# Autodesk Inventor assembly: Montagem1
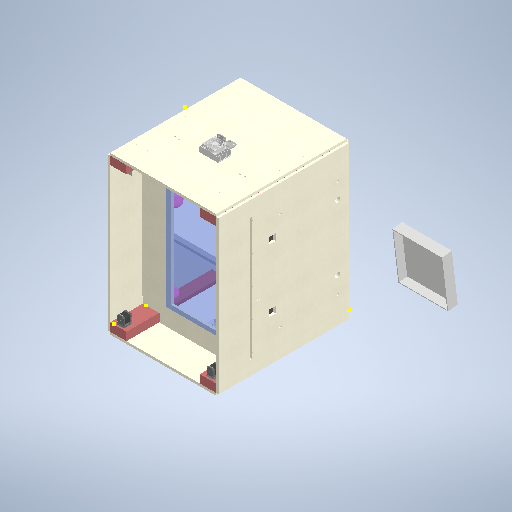
[picture p0: Inventor's stored thumbnail of the model, 512x512]
Saved by Autodesk Inventor 2025.1 (Build 291241000, 241)
## iProperties
Created: 2024-11-05
Part Number: Montagem1
Document SubType Name: Assembly
Designer: pedro
Author: pedro
## Documents named in this file (10)
- C:\Users\pedro\Documents\1-CoisasSerias\UTFPR\2024-2\Oficina\Estrutura\Montagem1 - Copia.iam
- C:\Users\pedro\Documents\1-CoisasSerias\UTFPR\2024-2\Oficina\Estrutura\estrutura2.ipt
- C:\Users\pedro\Documents\1-CoisasSerias\UTFPR\2024-2\Oficina\Estrutura\Pecas Prontas\Fan\Generic 7015 axial fan simplified\Generic 7015 axial fan simplified\cooler 40x40.ipt
- C:\Users\pedro\Documents\1-CoisasSerias\UTFPR\2024-2\Oficina\Estrutura\Pecas Prontas\Let light\Soquete\Soquete para lâmpada E27 MT-2302 - DECORLUX\Soquete para lâmpada E27 MT-2302 - DECORLUX\Soquete para lâmpad.iam
- C:\Users\pedro\Documents\1-CoisasSerias\UTFPR\2024-2\Oficina\Estrutura\step mother.iam
- C:\Users\pedro\Documents\1-CoisasSerias\UTFPR\2024-2\Oficina\Estrutura\Pecas Prontas\peltier\75W Peltier Air Cooler Kit 12V (TEC1-12706) - WiMas\75W Peltier Air Cooler Kit 12V (TEC1-12706) - WiMas\75W Peltier A.iam
- C:\Users\pedro\Documents\1-CoisasSerias\UTFPR\2024-2\Oficina\Estrutura\Pecas Prontas\peltier\step\L Bracket\L Bracket\L Bracket.ipt
- C:\Users\pedro\Documents\1-CoisasSerias\UTFPR\2024-2\Oficina\Estrutura\Pecas Prontas\reservatorio.ipt
- C:\Users\pedro\Documents\1-CoisasSerias\UTFPR\2024-2\Oficina\Estrutura\Pecas Prontas\vaso.ipt
- C:\Users\pedro\Documents\1-CoisasSerias\UTFPR\2024-2\Oficina\Estrutura\Pecas Prontas\temp\nema17-mounting-l-bracket-1.snapshot.2\NEMA17MountingLBracket.ipt
## Components (27 placed, 9 different names)
1. estrutura2:1 — Alinhado:1, Ângulo:1, Alinhado:2, Alinhado:3, Coincidente:1, Ângulo:2, Coincidente:2, Ângulo:3, Coincidente:12, Coincidente:13, Coincidente:14, Coincidente:15, Coincidente:18, Coincidente:19, Coincidente:20, Coincidente:21, Coincidente:22, Coincidente:26, Coincidente:27, Coincidente:28, Coincidente:29, Coincidente:31, Coincidente:32, Coincidente:33, Coincidente:34, Coincidente:35, Coincidente:36, Coincidente:37, Coincidente:38, Coincidente:39, Coincidente:40, Coincidente:41, Coincidente:42, Coincidente:43, Coincidente:44, Coincidente:45, Coincidente:46, Coincidente:47, Coincidente:48, Coincidente:49, Coincidente:50, Coincidente:51, Coincidente:52, Coincidente:53, Coincidente:54, Coincidente:55, Coincidente:56, Coincidente:57, Coincidente:58, Coincidente:59
2. cooler 40x40:1 — Alinhado:1, Ângulo:1, Alinhado:2, Alinhado:3
3. cooler 40x40:2
4. cooler 40x40:3
5. cooler 40x40:4
6. Soquete para lâmpad:2 [sub-assembly] — Coincidente:38, Coincidente:39
7. Soquete para lâmpad:3 [sub-assembly] — Coincidente:40, Coincidente:41
8. Soquete para lâmpad:4 [sub-assembly] — Coincidente:36, Coincidente:37
9. Soquete para lâmpad:8 [sub-assembly] — Coincidente:12, Coincidente:13, Coincidente:45
10. Soquete para lâmpad:9 [sub-assembly] — Coincidente:14, Coincidente:15, Coincidente:44
11. Soquete para lâmpad:10 [sub-assembly] — Coincidente:42, Coincidente:43
12. step mother:1 [sub-assembly] — Coincidente:18, Coincidente:19, Coincidente:20, Coincidente:21, Coincidente:22
13. step mother:3 [sub-assembly] — Coincidente:52
14. 75W Peltier A:1 [sub-assembly] — Coincidente:26, Coincidente:27
15. 75W Peltier A:2 [sub-assembly] — Coincidente:28, Coincidente:29, Coincidente:30
16. L Bracket:1 — Coincidente:30, Coincidente:31
17. L Bracket:2 — Coincidente:32
18. reservatorio:1
19. vaso:1 — Coincidente:33, Coincidente:34, Coincidente:35
20. vaso:2
21. L Bracket:3 — Coincidente:46
22. L Bracket:4 — Coincidente:47, Coincidente:48, Coincidente:49
23. L Bracket:5 — Coincidente:50
24. L Bracket:6 — Coincidente:51
25. step mother:4 [sub-assembly] — Coincidente:53
26. NEMA17MountingLBracket:1 — Coincidente:54, Coincidente:55, Coincidente:56
27. NEMA17MountingLBracket:2 — Coincidente:57, Coincidente:58, Coincidente:59
## Relationships (51: Mate 45, Flush 3, Angle 3)
- Alinhado:1 [Flush] (15 mm): estrutura2:1 ↔ cooler 40x40:1
- Ângulo:1 [Angle] (0 deg): estrutura2:1 ↔ cooler 40x40:1
- Alinhado:2 [Flush] (270 mm): estrutura2:1 ↔ cooler 40x40:1
- Alinhado:3 [Flush] (310 mm): estrutura2:1 ↔ cooler 40x40:1
- Coincidente:1 [Mate]: estrutura2:1
- Ângulo:2 [Angle] (0 deg): estrutura2:1
- Coincidente:2 [Mate]: estrutura2:1
- Ângulo:3 [Angle] (0 deg): estrutura2:1
- Coincidente:12 [Mate]: estrutura2:1 ↔ Soquete para lâmpad:8
- Coincidente:13 [Mate]: estrutura2:1 ↔ Soquete para lâmpad:8
- Coincidente:14 [Mate]: estrutura2:1 ↔ Soquete para lâmpad:9
- Coincidente:15 [Mate]: estrutura2:1 ↔ Soquete para lâmpad:9
- Coincidente:18 [Mate]: estrutura2:1 ↔ step mother:1
- Coincidente:19 [Mate]: estrutura2:1 ↔ step mother:1
- Coincidente:20 [Mate]: estrutura2:1 ↔ step mother:1
- Coincidente:21 [Mate]: estrutura2:1 ↔ step mother:1
- Coincidente:22 [Mate]: estrutura2:1 ↔ step mother:1
- Coincidente:26 [Mate]: estrutura2:1 ↔ 75W Peltier A:1
- Coincidente:27 [Mate]: estrutura2:1 ↔ 75W Peltier A:1
- Coincidente:28 [Mate]: estrutura2:1 ↔ 75W Peltier A:2
- Coincidente:29 [Mate]: estrutura2:1 ↔ 75W Peltier A:2
- Coincidente:30 [Mate]: 75W Peltier A:2 ↔ L Bracket:1
- Coincidente:31 [Mate]: estrutura2:1 ↔ L Bracket:1
- Coincidente:32 [Mate]: estrutura2:1 ↔ L Bracket:2
- Coincidente:33 [Mate]: estrutura2:1 ↔ vaso:1
- Coincidente:34 [Mate] (192.5 mm): estrutura2:1 ↔ vaso:1
- Coincidente:35 [Mate] (97.5 mm): estrutura2:1 ↔ vaso:1
- Coincidente:36 [Mate]: estrutura2:1 ↔ Soquete para lâmpad:4
- Coincidente:37 [Mate]: estrutura2:1 ↔ Soquete para lâmpad:4
- Coincidente:38 [Mate]: estrutura2:1 ↔ Soquete para lâmpad:2
- Coincidente:39 [Mate]: estrutura2:1 ↔ Soquete para lâmpad:2
- Coincidente:40 [Mate]: estrutura2:1 ↔ Soquete para lâmpad:3
- Coincidente:41 [Mate]: estrutura2:1 ↔ Soquete para lâmpad:3
- Coincidente:42 [Mate]: estrutura2:1 ↔ Soquete para lâmpad:10
- Coincidente:43 [Mate]: estrutura2:1 ↔ Soquete para lâmpad:10
- Coincidente:44 [Mate]: estrutura2:1 ↔ Soquete para lâmpad:9
- Coincidente:45 [Mate]: estrutura2:1 ↔ Soquete para lâmpad:8
- Coincidente:46 [Mate]: estrutura2:1 ↔ L Bracket:3
- Coincidente:47 [Mate]: estrutura2:1 ↔ L Bracket:4
- Coincidente:48 [Mate]: estrutura2:1 ↔ L Bracket:4
- Coincidente:49 [Mate]: estrutura2:1 ↔ L Bracket:4
- Coincidente:50 [Mate]: estrutura2:1 ↔ L Bracket:5
- Coincidente:51 [Mate]: estrutura2:1 ↔ L Bracket:6
- Coincidente:52 [Mate]: estrutura2:1 ↔ step mother:3
- Coincidente:53 [Mate]: estrutura2:1 ↔ step mother:4
- Coincidente:54 [Mate]: estrutura2:1 ↔ NEMA17MountingLBracket:1
- Coincidente:55 [Mate]: estrutura2:1 ↔ NEMA17MountingLBracket:1
- Coincidente:56 [Mate]: estrutura2:1 ↔ NEMA17MountingLBracket:1
- Coincidente:57 [Mate]: estrutura2:1 ↔ NEMA17MountingLBracket:2
- Coincidente:58 [Mate]: estrutura2:1 ↔ NEMA17MountingLBracket:2
- Coincidente:59 [Mate]: estrutura2:1 ↔ NEMA17MountingLBracket:2
